# Autodesk Inventor assembly: vslot-belt
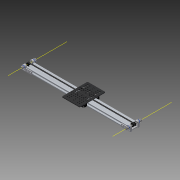
[picture p0: Inventor's stored thumbnail of the model, 180x180]
Saved by Autodesk Inventor 2015 (Build 190159000, 159)
## iProperties
Created: 2013-07-07
Part Number: vslot-belt
Document SubType Name: Assembly
Designer: mhgreen
Author: mhgreen
## Documents named in this file (6)
- C:\Users\Michael\Dropbox\autocad\openbuild\vslot-belt.iam
- C:\Users\Michael\Dropbox\autocad\openbuild\end-support-assembly.iam
- C:\Users\Michael\Dropbox\autocad\openbuild\makerslide-belt\Design Accelerator\Shaft1.iam
- C:\Users\Michael\Dropbox\autocad\openbuild\makerslide-belt\Design Accelerator\Synchronous Belts Transmission1.iam
- C:\Users\Michael\Dropbox\autocad\openbuild\parts\vslot_20x40x500.ipt
- C:\Users\Michael\Dropbox\autocad\openbuild\standard-vslot-plate.iam
## Components (6 placed, 5 different names)
1. end-support-assembly:1 [sub-assembly] — Mate:1, Mate:2, Flush:1, Flush:2
2. end-support-assembly:2 [sub-assembly] — Insert:1, Flush:3, Flush:4, Mate:3, Mate:4
3. 80mm shaft [sub-assembly] — Insert:1, Insert:2
4. Synchronous Belts Transmission:1 [sub-assembly] — Insert:2
5. extrusion_20x40x500:1 — Mate:1, Mate:2, Flush:1, Flush:2, Flush:3, Flush:4, Mate:3, Mate:4, Tangent:1, Tangent:2, Tangent:3, Tangent:4
6. standard-vslot-plate:1 [sub-assembly] — Tangent:1, Tangent:2, Tangent:3, Tangent:4
## Relationships (14: Mate 4, Flush 4, Tangent 4, Insert 2)
- Insert:1 (-76.75 mm): end-support-assembly:2 ↔ 80mm shaft
- Mate:1: end-support-assembly:1 ↔ extrusion_20x40x500:1
- Mate:2: end-support-assembly:1 ↔ extrusion_20x40x500:1
- Flush:1: end-support-assembly:1 ↔ extrusion_20x40x500:1
- Flush:2: end-support-assembly:1 ↔ extrusion_20x40x500:1
- Flush:3: end-support-assembly:2 ↔ extrusion_20x40x500:1
- Flush:4: end-support-assembly:2 ↔ extrusion_20x40x500:1
- Mate:3: end-support-assembly:2 ↔ extrusion_20x40x500:1
- Mate:4: end-support-assembly:2 ↔ extrusion_20x40x500:1
- Insert:2 (-45 mm): 80mm shaft ↔ Synchronous Belts Transmission:1
- Tangent:1: extrusion_20x40x500:1 ↔ standard-vslot-plate:1
- Tangent:2: extrusion_20x40x500:1 ↔ standard-vslot-plate:1
- Tangent:3: extrusion_20x40x500:1 ↔ standard-vslot-plate:1
- Tangent:4: extrusion_20x40x500:1 ↔ standard-vslot-plate:1
